# Autodesk Inventor assembly: E003_BoitierEcran
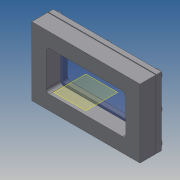
[picture p0: Inventor's stored thumbnail of the model, 180x180]
Saved by Autodesk Inventor 2021.3 (Build 253353000, 353)
## iProperties
Created: 2021-11-12
Part Number: E003_BoitierEcran
Document SubType Name: Assembly
Designer: gabri
Author: gabri
## Documents named in this file (6)
- D:\PGA\E003_BoitierEcran.iam
- D:\PGA\P018_BasEcranProtecLidar.ipt
- D:\PGA\P019_EcranProtecLidar.ipt
- D:\PGA\P020_Joint.ipt
- D:\PGA\P021_HautEcranProtecLidar.ipt
- C:\Users\gabri\Documents\Inventor\Content Center Files\R2021\en-US\ANSI B18.3.4M(1)\ANSI B18.3.4M - M3 x 0.5 x 10(2).ipt
## Components (12 placed, 5 different names)
1. P018_BasEcranProtecLidar:1 — Mate:1, Mate:2, Mate:3, Tangent:1, Tangent:2, Tangent:3, Tangent:4, Mate:4, Mate:5, Mate:7, Mate:8
2. P019_EcranProtecLidar:1 — Tangent:5, Mate:4, Mate:5, Mate:6
3. P020_Joint:1 — Tangent:1, Tangent:2, Tangent:3, Tangent:4, Tangent:5
4. P021_HautEcranProtecLidar:1 — Mate:6, Mate:7, Mate:8, Insert:1, Insert:2, Insert:3, Insert:4, Insert:5, Insert:6, Insert:7, Insert:8
5. Broached Hexagon Socket Button Head Cap Screw - Metric M3 x 0.5 x 10:1 — Insert:1
6. Broached Hexagon Socket Button Head Cap Screw - Metric M3 x 0.5 x 10:2 — Insert:2
7. Broached Hexagon Socket Button Head Cap Screw - Metric M3 x 0.5 x 10:3 — Insert:3
8. Broached Hexagon Socket Button Head Cap Screw - Metric M3 x 0.5 x 10:4 — Insert:4
9. Broached Hexagon Socket Button Head Cap Screw - Metric M3 x 0.5 x 10:5 — Insert:5
10. Broached Hexagon Socket Button Head Cap Screw - Metric M3 x 0.5 x 10:6 — Insert:6
11. Broached Hexagon Socket Button Head Cap Screw - Metric M3 x 0.5 x 10:7 — Insert:7
12. Broached Hexagon Socket Button Head Cap Screw - Metric M3 x 0.5 x 10:8 — Insert:8
## Relationships (21: Mate 8, Insert 8, Tangent 5)
- Mate:1: P018_BasEcranProtecLidar:1
- Mate:2: P018_BasEcranProtecLidar:1
- Mate:3: P018_BasEcranProtecLidar:1
- Tangent:1: P018_BasEcranProtecLidar:1 ↔ P020_Joint:1
- Tangent:2: P018_BasEcranProtecLidar:1 ↔ P020_Joint:1
- Tangent:3: P018_BasEcranProtecLidar:1 ↔ P020_Joint:1
- Tangent:4: P018_BasEcranProtecLidar:1 ↔ P020_Joint:1
- Tangent:5: P019_EcranProtecLidar:1 ↔ P020_Joint:1
- Mate:4: P018_BasEcranProtecLidar:1 ↔ P019_EcranProtecLidar:1
- Mate:5: P018_BasEcranProtecLidar:1 ↔ P019_EcranProtecLidar:1
- Mate:6: P019_EcranProtecLidar:1 ↔ P021_HautEcranProtecLidar:1
- Mate:7: P018_BasEcranProtecLidar:1 ↔ P021_HautEcranProtecLidar:1
- Mate:8: P018_BasEcranProtecLidar:1 ↔ P021_HautEcranProtecLidar:1
- Insert:1: P021_HautEcranProtecLidar:1 ↔ Broached Hexagon Socket Button Head Cap Screw - Metric M3 x 0.5 x 10:1
- Insert:2: P021_HautEcranProtecLidar:1 ↔ Broached Hexagon Socket Button Head Cap Screw - Metric M3 x 0.5 x 10:2
- Insert:3: P021_HautEcranProtecLidar:1 ↔ Broached Hexagon Socket Button Head Cap Screw - Metric M3 x 0.5 x 10:3
- Insert:4: P021_HautEcranProtecLidar:1 ↔ Broached Hexagon Socket Button Head Cap Screw - Metric M3 x 0.5 x 10:4
- Insert:5: P021_HautEcranProtecLidar:1 ↔ Broached Hexagon Socket Button Head Cap Screw - Metric M3 x 0.5 x 10:5
- Insert:6: P021_HautEcranProtecLidar:1 ↔ Broached Hexagon Socket Button Head Cap Screw - Metric M3 x 0.5 x 10:6
- Insert:7: P021_HautEcranProtecLidar:1 ↔ Broached Hexagon Socket Button Head Cap Screw - Metric M3 x 0.5 x 10:7
- Insert:8: P021_HautEcranProtecLidar:1 ↔ Broached Hexagon Socket Button Head Cap Screw - Metric M3 x 0.5 x 10:8
